# Autodesk Inventor assembly: sla2216
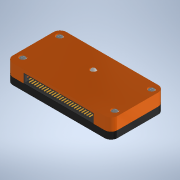
[picture p0: Inventor's stored thumbnail of the model, 180x180]
Saved by Autodesk Inventor 2021 (Build 250183000, 183)
## iProperties
Created: 2022-04-04
Part Number: sla2216
Document SubType Name: Assembly
Designer: Staňa
Author: Staňa
## Documents named in this file (7)
- D:\Projects\Hardware\sla2216\mech\sla2216.iam
- D:\Projects\Hardware\sla2216\mech\97790603111 (rev1).ipt
- D:\Projects\Hardware\sla2216\mech\sla2216.ipt
- D:\Projects\Hardware\sla2216\mech\casing-bot.ipt
- D:\Projects\Hardware\sla2216\mech\casing-top.ipt
- D:\Projects\Hardware\sla2216\mech\m3x05_thread_insert.ipt
- D:\Projects\Hardware\sla2216\mech\971080365 (rev1).ipt
## Components (15 placed, 6 different names)
1. sla2216-pcb:1 — Flush:1, Flush:2, Flush:3, Rotational:5, Rotational:6, Rotational:7, Rotational:8
2. casing-bot:1 — Rotational:1, Rotational:2, Rotational:3, Rotational:4
3. casing-top:1 — Rotational:9, Rotational:10, Rotational:11, Rotational:12
4. m3x05_thread_insert:1 — Rotational:1
5. m3x05_thread_insert:2 — Rotational:2
6. m3x05_thread_insert:3 — Rotational:3
7. m3x05_thread_insert:4 — Rotational:4
8. 971080365 (rev1):1 — Rotational:5
9. 971080365 (rev1):2 — Rotational:6
10. 971080365 (rev1):3 — Rotational:7
11. 971080365 (rev1):4 — Rotational:8
12. 97790603111 (rev1):1 — Rotational:9
13. 97790603111 (rev1):2 — Rotational:10
14. 97790603111 (rev1):3 — Rotational:11
15. 97790603111 (rev1):4 — Rotational:12
## Relationships (15: RevoluteJoint 12, Flush 3)
- Flush:1: sla2216-pcb:1
- Flush:2: sla2216-pcb:1
- Flush:3: sla2216-pcb:1
- Rotational:1 [RevoluteJoint]: casing-bot:1 ↔ m3x05_thread_insert:1
- Rotational:2 [RevoluteJoint]: casing-bot:1 ↔ m3x05_thread_insert:2
- Rotational:3 [RevoluteJoint]: casing-bot:1 ↔ m3x05_thread_insert:3
- Rotational:4 [RevoluteJoint]: casing-bot:1 ↔ m3x05_thread_insert:4
- Rotational:5 [RevoluteJoint]: sla2216-pcb:1 ↔ 971080365 (rev1):1
- Rotational:6 [RevoluteJoint]: sla2216-pcb:1 ↔ 971080365 (rev1):2
- Rotational:7 [RevoluteJoint]: sla2216-pcb:1 ↔ 971080365 (rev1):3
- Rotational:8 [RevoluteJoint]: sla2216-pcb:1 ↔ 971080365 (rev1):4
- Rotational:9 [RevoluteJoint]: casing-top:1 ↔ 97790603111 (rev1):1
- Rotational:10 [RevoluteJoint]: casing-top:1 ↔ 97790603111 (rev1):2
- Rotational:11 [RevoluteJoint]: casing-top:1 ↔ 97790603111 (rev1):3
- Rotational:12 [RevoluteJoint]: casing-top:1 ↔ 97790603111 (rev1):4
